# Autodesk Inventor assembly: TR08
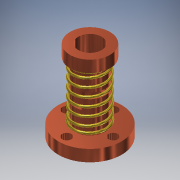
[picture p0: Inventor's stored thumbnail of the model, 180x180]
Saved by Autodesk Inventor 2017 SP1 (Build 210196100, 196)
## iProperties
Part Number: TR08
Material: Ogólny
Document SubType Name: Assembly
Designer: user
Author: user
## Documents named in this file (4)
- E:\OneDrive\Uczelnia\Zajęcia-prowadzone\2016-2017\KPG - Drukarka\TR08.iam
- E:\OneDrive\Uczelnia\Zajęcia-prowadzone\2016-2017\KPG - Drukarka\nakretka tr08.ipt
- E:\OneDrive\Uczelnia\Zajęcia-prowadzone\2016-2017\KPG - Drukarka\napinacz nakretki tr8.ipt
- E:\OneDrive\Uczelnia\Zajęcia-prowadzone\2016-2017\KPG - Drukarka\sprezyna nakretka tr 8.ipt
## Components (3 placed, 3 different names)
1. nakretka tr08:1 — Zestawiający:2, Zestawiający:3, Równoległy:1, Równoległy:2, Równoległy:3
2. napinacz nakretki tr8:1 — Zestawiający:1, Zestawiający:2, Zestawiający:3, Zestawiający:4
3. sprezyna nakretka tr 8:1 — Zestawiający:1, Zestawiający:4, Równoległy:1, Równoległy:2, Równoległy:3
## Relationships (7: Mate 4, Flush 3)
- Zestawiający:1 [Mate]: napinacz nakretki tr8:1 ↔ sprezyna nakretka tr 8:1
- Zestawiający:2 [Mate]: nakretka tr08:1 ↔ napinacz nakretki tr8:1
- Zestawiający:3 [Mate]: nakretka tr08:1 ↔ napinacz nakretki tr8:1
- Zestawiający:4 [Mate]: napinacz nakretki tr8:1 ↔ sprezyna nakretka tr 8:1
- Równoległy:1 [Flush]: nakretka tr08:1 ↔ sprezyna nakretka tr 8:1
- Równoległy:2 [Flush]: nakretka tr08:1 ↔ sprezyna nakretka tr 8:1
- Równoległy:3 [Flush]: nakretka tr08:1 ↔ sprezyna nakretka tr 8:1
